# Autodesk Inventor assembly: Basic Horiozontal Assembly
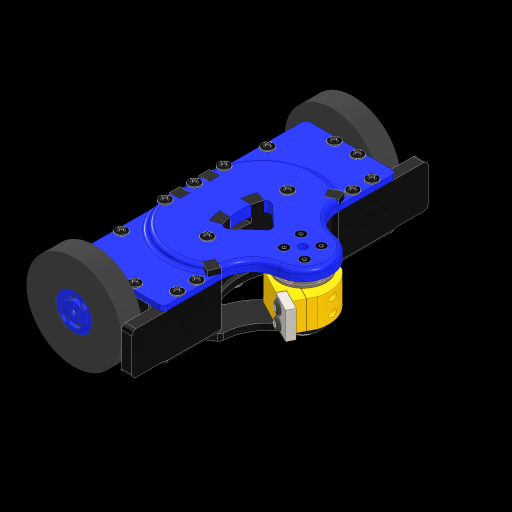
[picture p0: Inventor's stored thumbnail of the model, 512x512]
Saved by Autodesk Inventor 2023 (Build 270158000, 158)
## iProperties
Created: 2022-07-28
Part Number: Basic Horiozontal Assembly
Document SubType Name: Assembly
Designer: tandu
Mass: 379.783 g
Surface Area: 1215.62 cm^2
Volume: 265.888 cm^3
Density: 1.42836 g/cm^3
Author: tandu
## Documents named in this file (12)
- C:\Users\tandu\Documents\GrabCAD\Combat Robot Kits\To Sell\2WD Horizontal Mid Cutter\Inventor CAD Source Files\Basic Horiozontal Assembly.iam
- C:\Users\tandu\Documents\GrabCAD\Combat Robot Kits\To Sell\2WD Horizontal Mid Cutter\Inventor CAD Source Files\Horizontal TPU 22 Chassis.ipt
- C:\Users\tandu\Documents\GrabCAD\Combat Robot Kits\To Sell\2WD Horizontal Mid Cutter\Inventor CAD Source Files\FingerTech_Silver_Spark_223350.ipt
- C:\Users\tandu\Documents\GrabCAD\Combat Robot Kits\To Sell\2WD Horizontal Mid Cutter\Inventor CAD Source Files\BearingUpright.ipt
- C:\Users\tandu\Documents\GrabCAD\Combat Robot Kits\To Sell\2WD Horizontal Mid Cutter\Inventor CAD Source Files\LidAndMotorUpright.ipt
- C:\Users\tandu\Documents\GrabCAD\Combat Robot Kits\To Sell\2WD Horizontal Mid Cutter\Inventor CAD Source Files\300mAh 3S Lumenier Battery Mockup.ipt
- C:\Users\tandu\Documents\GrabCAD\Combat Robot Kits\To Sell\2WD Horizontal Mid Cutter\Inventor CAD Source Files\ClampDrum\D2822 Motor.ipt
- C:\Users\tandu\Documents\Inventor\Content Center Files\R2023\en-US\ISO 10642(2)\ISO 10642  - M3  x  8.ipt
- C:\Users\tandu\Documents\GrabCAD\Combat Robot Kits\To Sell\2WD Horizontal Mid Cutter\Inventor CAD Source Files\2 25 in x 0 50 in FT Wheel.ipt
- C:\Users\tandu\Documents\GrabCAD\Combat Robot Kits\To Sell\2WD Horizontal Mid Cutter\Inventor CAD Source Files\4 x 8 x 8 mm Needle Bearing Mockup.ipt
- C:\Users\tandu\Documents\GrabCAD\Combat Robot Kits\To Sell\2WD Horizontal Mid Cutter\Inventor CAD Source Files\ClampDrum\ClampDrumAssembly.iam
- C:\Users\tandu\Documents\GrabCAD\Combat Robot Kits\To Sell\2WD Horizontal Mid Cutter\Inventor CAD Source Files\90417A126_Phillips Rounded Head Thread-Forming Screws.ipt
## Components (35 placed, 11 different names)
1. Horizontal TPU 22 Chassis:1 — Insert:2, Mate:6, Insert:3, Mate:7, Mate:14, Angle:1, Angle:2, Mate:16, Flush:3, Mate:17, Mate:18, Mate:19, Flush:4, Flush:5
2. 2 25 in x 0 50 in FT Wheel:1
3. FingerTech_Silver_Spark_223350:1 — Insert:2, Mate:6
4. BearingUpright:1 — Mate:14, Angle:1, Flush:3, Mate:19, Insert:29, Insert:30, Insert:31, Insert:32, Insert:33
5. LidAndMotorUpright:1 — Angle:2, Mate:16, Flush:4, Flush:5, Insert:8, Insert:9, Insert:10, Insert:11, Insert:12, Insert:13, Insert:14, Insert:15, Insert:16, Insert:17, Insert:18, Insert:19, Insert:20, Insert:21, Insert:22, Insert:23, Insert:24, Insert:25, Insert:26, Insert:27, Insert:28
6. FingerTech_Silver_Spark_223350:2 — Insert:3, Mate:7
7. 2 25 in x 0 50 in FT Wheel:2
8. 300mAh 3S Lumenier Battery Mockup:1 — Mate:17, Mate:18
9. D2822 Motor:1 — Insert:6, Insert:7, Insert:8, Insert:9
10. 4 x 8 x 8 mm Needle Bearing Mockup:1 — Insert:7
11. ClampDrumAssembly:1 [sub-assembly] — Insert:6
12. 90417A126_Phillips Rounded Head Thread-Forming Screws:15 — Insert:28
13. 90417A126_Phillips Rounded Head Thread-Forming Screws:16 — Insert:30
14. 90417A126_Phillips Rounded Head Thread-Forming Screws:17 — Insert:29
15. 90417A126_Phillips Rounded Head Thread-Forming Screws:18 — Insert:31
16. 90417A126_Phillips Rounded Head Thread-Forming Screws:19 — Insert:33
17. 90417A126_Phillips Rounded Head Thread-Forming Screws:20 — Insert:32
18. DIN EN ISO 10642 M3  x  8:1 — Insert:10
19. DIN EN ISO 10642 M3  x  8:2 — Insert:13
20. DIN EN ISO 10642 M3  x  8:3 — Insert:12
21. DIN EN ISO 10642 M3  x  8:4 — Insert:11
22. 90417A126_Phillips Rounded Head Thread-Forming Screws:1 — Insert:16
23. 90417A126_Phillips Rounded Head Thread-Forming Screws:2 — Insert:14
24. 90417A126_Phillips Rounded Head Thread-Forming Screws:3 — Insert:15
25. 90417A126_Phillips Rounded Head Thread-Forming Screws:4 — Insert:17
26. 90417A126_Phillips Rounded Head Thread-Forming Screws:5 — Insert:18
27. 90417A126_Phillips Rounded Head Thread-Forming Screws:6 — Insert:20
28. 90417A126_Phillips Rounded Head Thread-Forming Screws:7 — Insert:21
29. 90417A126_Phillips Rounded Head Thread-Forming Screws:8 — Insert:19
30. 90417A126_Phillips Rounded Head Thread-Forming Screws:9 — Insert:23
31. 90417A126_Phillips Rounded Head Thread-Forming Screws:10 — Insert:22
32. 90417A126_Phillips Rounded Head Thread-Forming Screws:11 — Insert:27
33. 90417A126_Phillips Rounded Head Thread-Forming Screws:12 — Insert:26
34. 90417A126_Phillips Rounded Head Thread-Forming Screws:13 — Insert:25
35. 90417A126_Phillips Rounded Head Thread-Forming Screws:14 — Insert:24
## Relationships (44: Insert 32, Mate 7, Flush 3, Angle 2)
- Insert:2: Horizontal TPU 22 Chassis:1 ↔ FingerTech_Silver_Spark_223350:1
- Mate:6: Horizontal TPU 22 Chassis:1 ↔ FingerTech_Silver_Spark_223350:1
- Insert:3: Horizontal TPU 22 Chassis:1 ↔ FingerTech_Silver_Spark_223350:2
- Mate:7: Horizontal TPU 22 Chassis:1 ↔ FingerTech_Silver_Spark_223350:2
- [Insert]: Horizontal TPU 22 Chassis:1 ↔ 2 25 in x 0 50 in FT Wheel:1
- [Insert]: Horizontal TPU 22 Chassis:1 ↔ 2 25 in x 0 50 in FT Wheel:2
- Mate:14: Horizontal TPU 22 Chassis:1 ↔ BearingUpright:1
- Angle:1 (0 deg): Horizontal TPU 22 Chassis:1 ↔ BearingUpright:1
- Angle:2 (0 deg): Horizontal TPU 22 Chassis:1 ↔ LidAndMotorUpright:1
- Mate:16: Horizontal TPU 22 Chassis:1 ↔ LidAndMotorUpright:1
- Flush:3: Horizontal TPU 22 Chassis:1 ↔ BearingUpright:1
- Mate:17: Horizontal TPU 22 Chassis:1 ↔ 300mAh 3S Lumenier Battery Mockup:1
- Mate:18: Horizontal TPU 22 Chassis:1 ↔ 300mAh 3S Lumenier Battery Mockup:1
- Mate:19: Horizontal TPU 22 Chassis:1 ↔ BearingUpright:1
- Flush:4: Horizontal TPU 22 Chassis:1 ↔ LidAndMotorUpright:1
- Flush:5: Horizontal TPU 22 Chassis:1 ↔ LidAndMotorUpright:1
- Insert:6: D2822 Motor:1 ↔ ClampDrumAssembly:1
- Insert:7: D2822 Motor:1 ↔ 4 x 8 x 8 mm Needle Bearing Mockup:1
- Insert:8: LidAndMotorUpright:1 ↔ D2822 Motor:1
- Insert:9: LidAndMotorUpright:1 ↔ D2822 Motor:1
- Insert:10: LidAndMotorUpright:1 ↔ DIN EN ISO 10642 M3  x  8:1
- Insert:11: LidAndMotorUpright:1 ↔ DIN EN ISO 10642 M3  x  8:4
- Insert:12: LidAndMotorUpright:1 ↔ DIN EN ISO 10642 M3  x  8:3
- Insert:13: LidAndMotorUpright:1 ↔ DIN EN ISO 10642 M3  x  8:2
- Insert:14: LidAndMotorUpright:1 ↔ 90417A126_Phillips Rounded Head Thread-Forming Screws:2
- Insert:15: LidAndMotorUpright:1 ↔ 90417A126_Phillips Rounded Head Thread-Forming Screws:3
- Insert:16: LidAndMotorUpright:1 ↔ 90417A126_Phillips Rounded Head Thread-Forming Screws:1
- Insert:17: LidAndMotorUpright:1 ↔ 90417A126_Phillips Rounded Head Thread-Forming Screws:4
- Insert:18: LidAndMotorUpright:1 ↔ 90417A126_Phillips Rounded Head Thread-Forming Screws:5
- Insert:19: LidAndMotorUpright:1 ↔ 90417A126_Phillips Rounded Head Thread-Forming Screws:8
- Insert:20: LidAndMotorUpright:1 ↔ 90417A126_Phillips Rounded Head Thread-Forming Screws:6
- Insert:21: LidAndMotorUpright:1 ↔ 90417A126_Phillips Rounded Head Thread-Forming Screws:7
- Insert:22: LidAndMotorUpright:1 ↔ 90417A126_Phillips Rounded Head Thread-Forming Screws:10
- Insert:23: LidAndMotorUpright:1 ↔ 90417A126_Phillips Rounded Head Thread-Forming Screws:9
- Insert:24: LidAndMotorUpright:1 ↔ 90417A126_Phillips Rounded Head Thread-Forming Screws:14
- Insert:25: LidAndMotorUpright:1 ↔ 90417A126_Phillips Rounded Head Thread-Forming Screws:13
- Insert:26: LidAndMotorUpright:1 ↔ 90417A126_Phillips Rounded Head Thread-Forming Screws:12
- Insert:27: LidAndMotorUpright:1 ↔ 90417A126_Phillips Rounded Head Thread-Forming Screws:11
- Insert:28: LidAndMotorUpright:1 ↔ 90417A126_Phillips Rounded Head Thread-Forming Screws:15
- Insert:29: BearingUpright:1 ↔ 90417A126_Phillips Rounded Head Thread-Forming Screws:17
- Insert:30: BearingUpright:1 ↔ 90417A126_Phillips Rounded Head Thread-Forming Screws:16
- Insert:31: BearingUpright:1 ↔ 90417A126_Phillips Rounded Head Thread-Forming Screws:18
- Insert:32: BearingUpright:1 ↔ 90417A126_Phillips Rounded Head Thread-Forming Screws:20
- Insert:33: BearingUpright:1 ↔ 90417A126_Phillips Rounded Head Thread-Forming Screws:19
